# Autodesk Inventor assembly: 393 Motor Without backplate
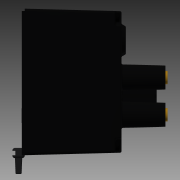
[picture p0: Inventor's stored thumbnail of the model, 180x180]
Saved by Autodesk Inventor 2016 SP2 (Build 200236200, 236)
## iProperties
Created: 2012-04-13
Part Number: 393 Motor Without backplate
Document SubType Name: Assembly
Designer: Phillip
Author: Phillip
## Documents named in this file (7)
- D:\Users\Owner\Desktop\Inventor Files\VEX Parts\Imperial\Motion\Components\393 Motor Without backplate.iam
- D:\Users\Owner\Desktop\Inventor Files\VEX Parts\Imperial\Motion\Components\SPPM206-0150BO.ipt
- D:\Users\Owner\Desktop\Inventor Files\VEX Parts\Imperial\Motion\Components\276-2177-002 Rev1.ipt
- D:\Users\Owner\Desktop\Inventor Files\VEX Parts\Imperial\Motion\Components\276-2177-003 Rev1.ipt
- D:\Users\Owner\Desktop\Inventor Files\VEX Parts\Imperial\Motion\Components\276-2177-018 Rev1.ipt
- D:\Users\Owner\Desktop\Inventor Files\VEX Parts\Imperial\Motion\Components\276-2177-019 Rev1.ipt
- D:\Users\Owner\Desktop\Inventor Files\VEX Parts\Imperial\Motion\Components\276-2177-008 Rev1.ipt
## Components (10 placed, 6 different names)
1. 276-2177-002 Rev1:1 — Mate:3, Flush:4, Mate:4
2. SPPM206-0150BO:1 — Insert:3
3. 276-2177-003 Rev1:1 — Insert:1, Insert:2, Insert:3, Insert:4, Flush:3, Mate:3, Flush:4, Mate:4, Mate:5, Mate:9, Mate:10, Flush:5, Flush:11
4. 276-2177-018 Rev1:1
5. SPPM206-0150BO:4 — Insert:2
6. 276-2177-019 Rev1:1 — Mate:10, Flush:11
7. 276-2177-019 Rev1:2 — Mate:9, Flush:5
8. SPPM206-0150BO:5 — Insert:4
9. SPPM206-0150BO:7 — Insert:1
10. 276-2177-008 Rev1:1 — Flush:3, Mate:5
## Relationships (13: Mate 5, Insert 4, Flush 4)
- Insert:1: 276-2177-003 Rev1:1 ↔ SPPM206-0150BO:7
- Insert:2: 276-2177-003 Rev1:1 ↔ SPPM206-0150BO:4
- Insert:3: SPPM206-0150BO:1 ↔ 276-2177-003 Rev1:1
- Insert:4: 276-2177-003 Rev1:1 ↔ SPPM206-0150BO:5
- Flush:3 (-0.0508 mm): 276-2177-003 Rev1:1 ↔ 276-2177-008 Rev1:1
- Mate:3: 276-2177-002 Rev1:1 ↔ 276-2177-003 Rev1:1
- Flush:4: 276-2177-002 Rev1:1 ↔ 276-2177-003 Rev1:1
- Mate:4: 276-2177-002 Rev1:1 ↔ 276-2177-003 Rev1:1
- Mate:5: 276-2177-003 Rev1:1 ↔ 276-2177-008 Rev1:1
- Mate:9: 276-2177-003 Rev1:1 ↔ 276-2177-019 Rev1:2
- Mate:10: 276-2177-003 Rev1:1 ↔ 276-2177-019 Rev1:1
- Flush:5 (0.7366 mm): 276-2177-003 Rev1:1 ↔ 276-2177-019 Rev1:2
- Flush:11 (0.7366 mm): 276-2177-003 Rev1:1 ↔ 276-2177-019 Rev1:1
